# Autodesk Inventor assembly: FanSetAssembly
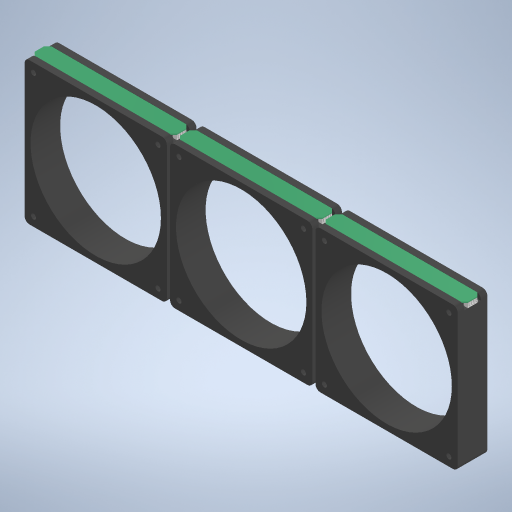
[picture p0: Inventor's stored thumbnail of the model, 512x512]
Saved by Autodesk Inventor 2023.1 (Build 271208000, 208)
## iProperties
Created: 2023-11-19
Part Number: FanSetAssembly
Document SubType Name: Assembly
Designer: Vinicius
Author: Vinicius
## Documents named in this file (3)
- D:\Git\WirelessCommunicationCoolingFans\Mechanical\FanSetAssembly.iam
- D:\Git\WirelessCommunicationCoolingFans\Mechanical\FanAssembly.iam
- FanAssembly.iam
## Components (3 placed, 1 different names)
1. FanAssembly:1 [sub-assembly] — Flush:1, Flush:3, Tangent:1
2. FanAssembly:2 [sub-assembly] — Flush:1, Flush:2, Flush:3, Flush:4, Tangent:1, Tangent:2
3. FanAssembly:3 [sub-assembly] — Flush:2, Flush:4, Tangent:2
## Relationships (6: Flush 4, Tangent 2)
- Flush:1: FanAssembly:1 ↔ FanAssembly:2
- Flush:2: FanAssembly:2 ↔ FanAssembly:3
- Flush:3: FanAssembly:1 ↔ FanAssembly:2
- Flush:4: FanAssembly:2 ↔ FanAssembly:3
- Tangent:1: FanAssembly:1 ↔ FanAssembly:2
- Tangent:2: FanAssembly:2 ↔ FanAssembly:3
